# Autodesk Inventor assembly: Intake - Mounting raiser
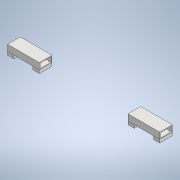
[picture p0: Inventor's stored thumbnail of the model, 180x180]
Saved by Autodesk Inventor 2020 (Build 240168000, 168)
## iProperties
Created: 2020-02-05
Part Number: Intake - Mounting raiser
Document SubType Name: Assembly
Designer: aidan
Author: aidan
## Documents named in this file (4)
- C:\Users\aidan\Desktop\T3 Robotics\CAD\Intake - Mounting raiser.iam
- C:\Users\aidan\Desktop\T3 Robotics\CAD\Intake - Lexan Raiser.ipt
- C:\Users\aidan\Desktop\T3 Robotics\CAD\Intake - Lexan Raiser  inner.ipt
- C:\Users\aidan\Desktop\T3 Robotics\CAD\Intake - 2 by 1 Aluminum Mounting CrossBar.ipt
## Components (3 placed, 3 different names)
1. Intake - Lexan Raiser:1 — Mate:1, Flush:1, Flush:2
2. Intake - Lexan Raiser  inner:1 — Mate:1, Flush:1, Flush:2, Flush:3, Flush:4, Mate:2
3. Intake - 2 by 1 Aluminum Mounting CrossBar:1 — Flush:3, Flush:4, Mate:2
## Relationships (6: Flush 4, Mate 2)
- Mate:1 (76.2 mm): Intake - Lexan Raiser:1 ↔ Intake - Lexan Raiser  inner:1
- Flush:1: Intake - Lexan Raiser:1 ↔ Intake - Lexan Raiser  inner:1
- Flush:2: Intake - Lexan Raiser:1 ↔ Intake - Lexan Raiser  inner:1
- Flush:3: Intake - Lexan Raiser  inner:1 ↔ Intake - 2 by 1 Aluminum Mounting CrossBar:1
- Flush:4: Intake - Lexan Raiser  inner:1 ↔ Intake - 2 by 1 Aluminum Mounting CrossBar:1
- Mate:2: Intake - Lexan Raiser  inner:1 ↔ Intake - 2 by 1 Aluminum Mounting CrossBar:1
